# Autodesk Inventor assembly: car
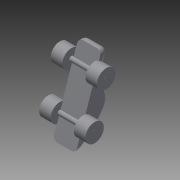
[picture p0: Inventor's stored thumbnail of the model, 180x180]
Saved by Autodesk Inventor 2015 (Build 190159000, 159)
## iProperties
Created: 2014-07-13
Part Number: car
Document SubType Name: Assembly
Designer: shohei
Author: shohei
## Documents named in this file (4)
- C:\Users\shohei\Documents\Inventor\FufuPounder\car.iam
- C:\Users\shohei\Documents\Inventor\FufuPounder\body.ipt
- C:\Users\shohei\Documents\Inventor\FufuPounder\driveshaft.ipt
- C:\Users\shohei\Documents\Inventor\FufuPounder\wheel.ipt
## Components (7 placed, 3 different names)
1. body:1 — Mate:1, Mate:2
2. driveshaft:1 — Mate:1, Rigid:1, Rotational:1
3. wheel:1 — Rotational:2
4. wheel:2 — Rigid:1
5. wheel:3 — Rotational:1
6. wheel:4 — Rigid:2
7. driveshaft:2 — Mate:2, Rotational:2, Rigid:2
## Relationships (6: Mate 2, WeldJoint 2, RevoluteJoint 2)
- Mate:1: body:1 ↔ driveshaft:1
- Mate:2: body:1 ↔ driveshaft:2
- Rigid:1 [WeldJoint]: driveshaft:1 ↔ wheel:2
- Rotational:1 [RevoluteJoint]: driveshaft:1 ↔ wheel:3
- Rotational:2 [RevoluteJoint]: wheel:1 ↔ driveshaft:2
- Rigid:2 [WeldJoint]: wheel:4 ↔ driveshaft:2
